# Autodesk Inventor assembly: RA-Manager_Controller
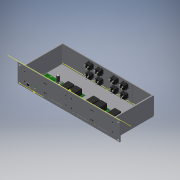
[picture p0: Inventor's stored thumbnail of the model, 180x180]
Saved by Autodesk Inventor 2019.4 (Build 234330000, 330)
## iProperties
Company: Open CASCADE
Created: 2020-03-09
Part Number: RA-Manager_Controller
Material: Genérico
Description: Open CASCADE Model
Document SubType Name: Assembly
Designer: caio.santos
Authority: Unknown
Title: Open CASCADE Shape Model
Author: Author
## Documents named in this file (38)
- C:\Users\caiom\Desktop\Ra-Manager_Mecanica\RA-Manager_Montagem.iam
- C:\Users\caiom\Desktop\Ra-Manager_Mecanica\Ra-Manager_Painel_Frontal.ipt
- C:\Users\caiom\Desktop\Ra-Manager_Mecanica\Ra-Manager_Base.ipt
- C:\Users\caiom\Desktop\Ra-Manager_Mecanica\Ra-Manager_Painel_Traseiro.ipt
- C:\Users\caiom\Desktop\Ra-Manager_Mecanica\Ra-Manager_Painel_Superior.ipt
- C:\Users\caiom\Desktop\Ra-Manager_Mecanica\Ra-Manager_Montagem_Controller.iam
- C:\Users\caiom\Desktop\Ra-Manager_Mecanica\Ra-Manager_Montagem_Relays.iam
- C:\Users\caiom\Desktop\Ra-Manager_Mecanica\Ra-Manager_Painel-Placas_Tras_Cego.ipt
- C:\Users\caiom\Desktop\Ra-Manager_Mecanica\Ra-Manager_Montagem_Plugs.iam
- C:\Users\caiom\Desktop\Ra-Manager_Mecanica\Espacador_Placas.ipt
- C:\Users\caiom\Desktop\Ra-Manager_Mecanica\RA-Manager_Montagem\Design Accelerator\Conexão aparafusada9.iam
- C:\Users\caiom\Desktop\Ra-Manager_Mecanica\RA-Manager_Montagem\Design Accelerator\Conexão aparafusada10.iam
- C:\Users\caiom\Desktop\Ra-Manager_Mecanica\RA-Manager_Montagem\Design Accelerator\Conexão aparafusada11.iam
- C:\Users\caiom\Desktop\Ra-Manager_Mecanica\RA-Manager_Montagem\Design Accelerator\Conexão aparafusada12.iam
- C:\Users\caiom\Desktop\Ra-Manager_Mecanica\RA-Manager_Montagem\Design Accelerator\Conexão aparafusada13.iam
- C:\Users\caiom\Desktop\Ra-Manager_Mecanica\RA-Manager_Montagem\Design Accelerator\Conexão aparafusada14.iam
- C:\Users\caiom\Desktop\Ra-Manager_Mecanica\RA-Manager_Montagem\Design Accelerator\Conexão aparafusada15.iam
- C:\Users\caiom\Desktop\Ra-Manager_Mecanica\RA-Manager_Montagem\Design Accelerator\Conexão aparafusada16.iam
- C:\Users\caiom\Desktop\Ra-Manager_Mecanica\RA-Manager_Montagem\Design Accelerator\Conexão aparafusada17.iam
- C:\Users\caiom\Desktop\Ra-Manager_Mecanica\RA-Manager_Montagem\Design Accelerator\Conexão aparafusada18.iam
- C:\Users\caiom\Desktop\Ra-Manager_Mecanica\RA-Manager_Montagem\Design Accelerator\Conexão aparafusada19.iam
- C:\Users\caiom\Desktop\Ra-Manager_Mecanica\RA-Manager_Montagem\Design Accelerator\Conexão aparafusada20.iam
- C:\Users\caiom\Desktop\Ra-Manager_Mecanica\RA-Manager_Montagem\Design Accelerator\Conexão aparafusada21.iam
- C:\Users\caiom\Desktop\Ra-Manager_Mecanica\RA-Manager_Montagem\Design Accelerator\Conexão aparafusada22.iam
- C:\Users\caiom\Desktop\Ra-Manager_Mecanica\RA-Manager_Montagem\Design Accelerator\Conexão aparafusada23.iam
- C:\Users\caiom\Desktop\Ra-Manager_Mecanica\RA-Manager_Montagem\Design Accelerator\Conexão aparafusada24.iam
- C:\Users\caiom\Desktop\Ra-Manager_Mecanica\RA-Manager_Montagem\Design Accelerator\Conexão aparafusada25.iam
- C:\Users\caiom\Desktop\Ra-Manager_Mecanica\RA-Manager_Montagem\Design Accelerator\Conexão aparafusada26.iam
- C:\Users\caiom\Desktop\Ra-Manager_Mecanica\RA-Manager_Montagem\Design Accelerator\Conexão aparafusada27.iam
- C:\Users\caiom\Desktop\Ra-Manager_Mecanica\RA-Manager_Montagem\Design Accelerator\Conexão aparafusada28.iam
- C:\Users\caiom\Desktop\Ra-Manager_Mecanica\RA-Manager_Montagem\Design Accelerator\Conexão aparafusada29.iam
- C:\Users\caiom\Desktop\Ra-Manager_Mecanica\RA-Manager_Montagem\Design Accelerator\Conexão aparafusada30.iam
- C:\Users\caiom\Desktop\Ra-Manager_Mecanica\RA-Manager_Montagem\Design Accelerator\Conexão aparafusada31.iam
- C:\Users\caiom\Desktop\Ra-Manager_Mecanica\RA-Manager_Montagem\Design Accelerator\Conexão aparafusada32.iam
- C:\Users\caiom\Desktop\Ra-Manager_Mecanica\RA-Manager_Montagem\Design Accelerator\Conexão aparafusada33.iam
- C:\Users\caiom\Desktop\Ra-Manager_Mecanica\RA-Manager_Montagem\Design Accelerator\Conexão aparafusada34.iam
- C:\Users\caiom\Desktop\Ra-Manager_Mecanica\RA-Manager_Montagem\Design Accelerator\Conexão aparafusada35.iam
- C:\Users\caiom\Desktop\Ra-Manager_Mecanica\RA-Manager_Montagem\Design Accelerator\Conexão aparafusada36.iam
## Components (56 placed, 10 different names)
1. Ra-Manager_Painel_Frontal:1 — Coincidência:3, Alinhamento:2, Coincidência:4, Alinhamento:7, Coincidência:12, Coincidência:16, Alinhamento:9, Coincidência:23, Coincidência:24, Coincidência:25, Coincidência:42, Coincidência:44, Coincidência:61, Coincidência:62, Coincidência:100, Coincidência:102, Coincidência:104, Coincidência:106, Coincidência:108, Coincidência:110, Coincidência:112, Coincidência:114, Coincidência:116, Coincidência:118, Coincidência:120, Coincidência:122
2. Ra-Manager_Base:1 — Alinhamento:2, Coincidência:4, Coincidência:7, Coincidência:10, Alinhamento:7, Alinhamento:8, Coincidência:13, Alinhamento:10, Alinhamento:11, Coincidência:29, Coincidência:49, Coincidência:50, Coincidência:51, Coincidência:52, Coincidência:53, Coincidência:54, Coincidência:55, Coincidência:56, Coincidência:57, Coincidência:58, Coincidência:59, Coincidência:60, Coincidência:63, Coincidência:64, Coincidência:65, Coincidência:66, Coincidência:67, Coincidência:68, Coincidência:69, Coincidência:70, Coincidência:71, Coincidência:72, Coincidência:73, Coincidência:74, Coincidência:75, Coincidência:76, Coincidência:77, Coincidência:78, Coincidência:79, Coincidência:80, Coincidência:81, Coincidência:82, Coincidência:83, Coincidência:84, Coincidência:85, Coincidência:86, Coincidência:87, Coincidência:88, Coincidência:89, Coincidência:90, Coincidência:91, Coincidência:92, Coincidência:93, Coincidência:94, Coincidência:95, Coincidência:96, Coincidência:97, Coincidência:98
3. Ra-Manager_Painel_Traseiro:1 — Alinhamento:10, Alinhamento:11, Coincidência:29, Coincidência:30, Coincidência:31, Coincidência:32, Coincidência:33, Coincidência:34, Coincidência:35, Coincidência:36, Coincidência:38, Coincidência:39, Coincidência:40, Coincidência:41
4. Ra-Manager_Painel_Superior:1 — Alinhamento:8, Coincidência:12, Coincidência:13
5. Ra-Manager_Montagem_Controller:1 [sub-assembly] — Alinhamento:9, Coincidência:61, Coincidência:62, Coincidência:99, Coincidência:101, Coincidência:103, Coincidência:105
6. Ra-Manager_Montagem_Relays:1 [sub-assembly] — Coincidência:16, Coincidência:107, Coincidência:109, Coincidência:111, Coincidência:113
7. Ra-Manager_Montagem_Relays:2 [sub-assembly] — Coincidência:23, Coincidência:24, Coincidência:25, Coincidência:43, Coincidência:115, Coincidência:117, Coincidência:119, Coincidência:121
8. Ra-Manager_Montagem_Relays:3 [sub-assembly] — Coincidência:42, Coincidência:43, Coincidência:44
9. Ra-Manager_Painel-Placas_Tras_Cego:1 — Coincidência:30, Coincidência:31, Coincidência:32, Coincidência:37
10. Ra-Manager_Montagem_Plugs:1 [sub-assembly] — Coincidência:33, Coincidência:34, Coincidência:35
11. Ra-Manager_Montagem_Plugs:2 [sub-assembly] — Coincidência:36, Coincidência:37, Coincidência:38
12. Ra-Manager_Painel-Placas_Tras_Cego:2 — Coincidência:39, Coincidência:40, Coincidência:41
13. Espacador_Placas:1 — Coincidência:64
14. Espacador_Placas:2 — Coincidência:65
15. Espacador_Placas:3 — Coincidência:66
16. Espacador_Placas:4 — Coincidência:63
17. Espacador_Placas:5 — Coincidência:52
18. Espacador_Placas:6 — Coincidência:49
19. Espacador_Placas:7 — Coincidência:51
20. Espacador_Placas:8 — Coincidência:50
21. Espacador_Placas:9 — Coincidência:56
22. Espacador_Placas:10 — Coincidência:54
23. Espacador_Placas:11 — Coincidência:55
24. Espacador_Placas:12 — Coincidência:53
25. Espacador_Placas:13 — Coincidência:59
26. Espacador_Placas:14 — Coincidência:57
27. Espacador_Placas:15 — Coincidência:60
28. Espacador_Placas:16 — Coincidência:58
29. Conexão aparafusada:1 [sub-assembly] — Coincidência:67, Coincidência:68
30. Conexão aparafusada:2 [sub-assembly] — Coincidência:69, Coincidência:70
31. Conexão aparafusada:3 [sub-assembly] — Coincidência:71, Coincidência:72
32. Conexão aparafusada:4 [sub-assembly] — Coincidência:73, Coincidência:74
33. Conexão aparafusada:5 [sub-assembly] — Coincidência:75, Coincidência:76
34. Conexão aparafusada:6 [sub-assembly] — Coincidência:77, Coincidência:78
35. Conexão aparafusada:7 [sub-assembly] — Coincidência:79, Coincidência:80
36. Conexão aparafusada:8 [sub-assembly] — Coincidência:81, Coincidência:82
37. Conexão aparafusada:9 [sub-assembly] — Coincidência:83, Coincidência:84
38. Conexão aparafusada:10 [sub-assembly] — Coincidência:85, Coincidência:86
39. Conexão aparafusada:11 [sub-assembly] — Coincidência:87, Coincidência:88
40. Conexão aparafusada:12 [sub-assembly] — Coincidência:89, Coincidência:90
41. Conexão aparafusada:13 [sub-assembly] — Coincidência:91, Coincidência:92
42. Conexão aparafusada:14 [sub-assembly] — Coincidência:93, Coincidência:94
43. Conexão aparafusada:15 [sub-assembly] — Coincidência:95, Coincidência:96
44. Conexão aparafusada:16 [sub-assembly] — Coincidência:97, Coincidência:98
45. Conexão aparafusada:17 [sub-assembly] — Coincidência:99, Coincidência:100
46. Conexão aparafusada:18 [sub-assembly] — Coincidência:101, Coincidência:102
47. Conexão aparafusada:19 [sub-assembly] — Coincidência:103, Coincidência:104
48. Conexão aparafusada:20 [sub-assembly] — Coincidência:105, Coincidência:106
49. Conexão aparafusada:21 [sub-assembly] — Coincidência:107, Coincidência:108
50. Conexão aparafusada:22 [sub-assembly] — Coincidência:109, Coincidência:110
51. Conexão aparafusada:23 [sub-assembly] — Coincidência:111, Coincidência:112
52. Conexão aparafusada:24 [sub-assembly] — Coincidência:113, Coincidência:114
53. Conexão aparafusada:25 [sub-assembly] — Coincidência:115, Coincidência:116
54. Conexão aparafusada:26 [sub-assembly] — Coincidência:117, Coincidência:118
55. Conexão aparafusada:27 [sub-assembly] — Coincidência:119, Coincidência:120
56. Conexão aparafusada:28 [sub-assembly] — Coincidência:121, Coincidência:122
## Relationships (107: Mate 101, Flush 6)
- Coincidência:3 [Mate]: Ra-Manager_Painel_Frontal:1
- Alinhamento:2 [Flush]: Ra-Manager_Painel_Frontal:1 ↔ Ra-Manager_Base:1
- Coincidência:4 [Mate]: Ra-Manager_Painel_Frontal:1 ↔ Ra-Manager_Base:1
- Coincidência:7 [Mate]: Ra-Manager_Base:1
- Coincidência:10 [Mate]: Ra-Manager_Base:1
- Coincidência:11 [Mate] (180 mm)
- Alinhamento:7 [Flush]: Ra-Manager_Painel_Frontal:1 ↔ Ra-Manager_Base:1
- Alinhamento:8 [Flush]: Ra-Manager_Base:1 ↔ Ra-Manager_Painel_Superior:1
- Coincidência:12 [Mate]: Ra-Manager_Painel_Frontal:1 ↔ Ra-Manager_Painel_Superior:1
- Coincidência:13 [Mate]: Ra-Manager_Base:1 ↔ Ra-Manager_Painel_Superior:1
- Coincidência:16 [Mate]: Ra-Manager_Painel_Frontal:1 ↔ Ra-Manager_Montagem_Relays:1
- Alinhamento:9 [Flush]: Ra-Manager_Painel_Frontal:1 ↔ Ra-Manager_Montagem_Controller:1
- Coincidência:23 [Mate]: Ra-Manager_Painel_Frontal:1 ↔ Ra-Manager_Montagem_Relays:2
- Coincidência:24 [Mate]: Ra-Manager_Painel_Frontal:1 ↔ Ra-Manager_Montagem_Relays:2
- Coincidência:25 [Mate]: Ra-Manager_Painel_Frontal:1 ↔ Ra-Manager_Montagem_Relays:2
- Alinhamento:10 [Flush]: Ra-Manager_Base:1 ↔ Ra-Manager_Painel_Traseiro:1
- Alinhamento:11 [Flush]: Ra-Manager_Base:1 ↔ Ra-Manager_Painel_Traseiro:1
- Coincidência:29 [Mate]: Ra-Manager_Base:1 ↔ Ra-Manager_Painel_Traseiro:1
- Coincidência:30 [Mate]: Ra-Manager_Painel_Traseiro:1 ↔ Ra-Manager_Painel-Placas_Tras_Cego:1
- Coincidência:31 [Mate]: Ra-Manager_Painel_Traseiro:1 ↔ Ra-Manager_Painel-Placas_Tras_Cego:1
- Coincidência:32 [Mate]: Ra-Manager_Painel_Traseiro:1 ↔ Ra-Manager_Painel-Placas_Tras_Cego:1
- Coincidência:33 [Mate]: Ra-Manager_Painel_Traseiro:1 ↔ Ra-Manager_Montagem_Plugs:1
- Coincidência:34 [Mate]: Ra-Manager_Painel_Traseiro:1 ↔ Ra-Manager_Montagem_Plugs:1
- Coincidência:35 [Mate]: Ra-Manager_Painel_Traseiro:1 ↔ Ra-Manager_Montagem_Plugs:1
- Coincidência:36 [Mate]: Ra-Manager_Painel_Traseiro:1 ↔ Ra-Manager_Montagem_Plugs:2
- Coincidência:37 [Mate]: Ra-Manager_Painel-Placas_Tras_Cego:1 ↔ Ra-Manager_Montagem_Plugs:2
- Coincidência:38 [Mate]: Ra-Manager_Painel_Traseiro:1 ↔ Ra-Manager_Montagem_Plugs:2
- Coincidência:39 [Mate]: Ra-Manager_Painel_Traseiro:1 ↔ Ra-Manager_Painel-Placas_Tras_Cego:2
- Coincidência:40 [Mate]: Ra-Manager_Painel_Traseiro:1 ↔ Ra-Manager_Painel-Placas_Tras_Cego:2
- Coincidência:41 [Mate]: Ra-Manager_Painel_Traseiro:1 ↔ Ra-Manager_Painel-Placas_Tras_Cego:2
- Coincidência:42 [Mate]: Ra-Manager_Painel_Frontal:1 ↔ Ra-Manager_Montagem_Relays:3
- Coincidência:43 [Mate]: Ra-Manager_Montagem_Relays:2 ↔ Ra-Manager_Montagem_Relays:3
- Coincidência:44 [Mate]: Ra-Manager_Painel_Frontal:1 ↔ Ra-Manager_Montagem_Relays:3
- Coincidência:49 [Mate]: Ra-Manager_Base:1 ↔ Espacador_Placas:6
- Coincidência:50 [Mate]: Ra-Manager_Base:1 ↔ Espacador_Placas:8
- Coincidência:51 [Mate]: Ra-Manager_Base:1 ↔ Espacador_Placas:7
- Coincidência:52 [Mate]: Ra-Manager_Base:1 ↔ Espacador_Placas:5
- Coincidência:53 [Mate]: Ra-Manager_Base:1 ↔ Espacador_Placas:12
- Coincidência:54 [Mate]: Ra-Manager_Base:1 ↔ Espacador_Placas:10
- Coincidência:55 [Mate]: Ra-Manager_Base:1 ↔ Espacador_Placas:11
- Coincidência:56 [Mate]: Ra-Manager_Base:1 ↔ Espacador_Placas:9
- Coincidência:57 [Mate]: Ra-Manager_Base:1 ↔ Espacador_Placas:14
- Coincidência:58 [Mate]: Ra-Manager_Base:1 ↔ Espacador_Placas:16
- Coincidência:59 [Mate]: Ra-Manager_Base:1 ↔ Espacador_Placas:13
- Coincidência:60 [Mate]: Ra-Manager_Base:1 ↔ Espacador_Placas:15
- Coincidência:61 [Mate]: Ra-Manager_Painel_Frontal:1 ↔ Ra-Manager_Montagem_Controller:1
- Coincidência:62 [Mate]: Ra-Manager_Painel_Frontal:1 ↔ Ra-Manager_Montagem_Controller:1
- Coincidência:63 [Mate]: Ra-Manager_Base:1 ↔ Espacador_Placas:4
- Coincidência:64 [Mate]: Ra-Manager_Base:1 ↔ Espacador_Placas:1
- Coincidência:65 [Mate]: Ra-Manager_Base:1 ↔ Espacador_Placas:2
- Coincidência:66 [Mate]: Ra-Manager_Base:1 ↔ Espacador_Placas:3
- Coincidência:67 [Mate]: Ra-Manager_Base:1 ↔ Conexão aparafusada:1
- Coincidência:68 [Mate]: Ra-Manager_Base:1 ↔ Conexão aparafusada:1
- Coincidência:69 [Mate]: Ra-Manager_Base:1 ↔ Conexão aparafusada:2
- Coincidência:70 [Mate]: Ra-Manager_Base:1 ↔ Conexão aparafusada:2
- Coincidência:71 [Mate]: Ra-Manager_Base:1 ↔ Conexão aparafusada:3
- Coincidência:72 [Mate]: Ra-Manager_Base:1 ↔ Conexão aparafusada:3
- Coincidência:73 [Mate]: Ra-Manager_Base:1 ↔ Conexão aparafusada:4
- Coincidência:74 [Mate]: Ra-Manager_Base:1 ↔ Conexão aparafusada:4
- Coincidência:75 [Mate]: Ra-Manager_Base:1 ↔ Conexão aparafusada:5
- Coincidência:76 [Mate]: Ra-Manager_Base:1 ↔ Conexão aparafusada:5
- Coincidência:77 [Mate]: Ra-Manager_Base:1 ↔ Conexão aparafusada:6
- Coincidência:78 [Mate]: Ra-Manager_Base:1 ↔ Conexão aparafusada:6
- Coincidência:79 [Mate]: Ra-Manager_Base:1 ↔ Conexão aparafusada:7
- Coincidência:80 [Mate]: Ra-Manager_Base:1 ↔ Conexão aparafusada:7
- Coincidência:81 [Mate]: Ra-Manager_Base:1 ↔ Conexão aparafusada:8
- Coincidência:82 [Mate]: Ra-Manager_Base:1 ↔ Conexão aparafusada:8
- Coincidência:83 [Mate]: Ra-Manager_Base:1 ↔ Conexão aparafusada:9
- Coincidência:84 [Mate]: Ra-Manager_Base:1 ↔ Conexão aparafusada:9
- Coincidência:85 [Mate]: Ra-Manager_Base:1 ↔ Conexão aparafusada:10
- Coincidência:86 [Mate]: Ra-Manager_Base:1 ↔ Conexão aparafusada:10
- Coincidência:87 [Mate]: Ra-Manager_Base:1 ↔ Conexão aparafusada:11
- Coincidência:88 [Mate]: Ra-Manager_Base:1 ↔ Conexão aparafusada:11
- Coincidência:89 [Mate]: Ra-Manager_Base:1 ↔ Conexão aparafusada:12
- Coincidência:90 [Mate]: Ra-Manager_Base:1 ↔ Conexão aparafusada:12
- Coincidência:91 [Mate]: Ra-Manager_Base:1 ↔ Conexão aparafusada:13
- Coincidência:92 [Mate]: Ra-Manager_Base:1 ↔ Conexão aparafusada:13
- Coincidência:93 [Mate]: Ra-Manager_Base:1 ↔ Conexão aparafusada:14
- Coincidência:94 [Mate]: Ra-Manager_Base:1 ↔ Conexão aparafusada:14
- Coincidência:95 [Mate]: Ra-Manager_Base:1 ↔ Conexão aparafusada:15
- Coincidência:96 [Mate]: Ra-Manager_Base:1 ↔ Conexão aparafusada:15
- Coincidência:97 [Mate]: Ra-Manager_Base:1 ↔ Conexão aparafusada:16
- Coincidência:98 [Mate]: Ra-Manager_Base:1 ↔ Conexão aparafusada:16
- Coincidência:99 [Mate]: Ra-Manager_Montagem_Controller:1 ↔ Conexão aparafusada:17
- Coincidência:100 [Mate]: Ra-Manager_Painel_Frontal:1 ↔ Conexão aparafusada:17
- Coincidência:101 [Mate]: Ra-Manager_Montagem_Controller:1 ↔ Conexão aparafusada:18
- Coincidência:102 [Mate]: Ra-Manager_Painel_Frontal:1 ↔ Conexão aparafusada:18
- Coincidência:103 [Mate]: Ra-Manager_Montagem_Controller:1 ↔ Conexão aparafusada:19
- Coincidência:104 [Mate]: Ra-Manager_Painel_Frontal:1 ↔ Conexão aparafusada:19
- Coincidência:105 [Mate]: Ra-Manager_Montagem_Controller:1 ↔ Conexão aparafusada:20
- Coincidência:106 [Mate]: Ra-Manager_Painel_Frontal:1 ↔ Conexão aparafusada:20
- Coincidência:107 [Mate]: Ra-Manager_Montagem_Relays:1 ↔ Conexão aparafusada:21
- Coincidência:108 [Mate]: Ra-Manager_Painel_Frontal:1 ↔ Conexão aparafusada:21
- Coincidência:109 [Mate]: Ra-Manager_Montagem_Relays:1 ↔ Conexão aparafusada:22
- Coincidência:110 [Mate]: Ra-Manager_Painel_Frontal:1 ↔ Conexão aparafusada:22
- Coincidência:111 [Mate]: Ra-Manager_Montagem_Relays:1 ↔ Conexão aparafusada:23
- Coincidência:112 [Mate]: Ra-Manager_Painel_Frontal:1 ↔ Conexão aparafusada:23
- Coincidência:113 [Mate]: Ra-Manager_Montagem_Relays:1 ↔ Conexão aparafusada:24
- Coincidência:114 [Mate]: Ra-Manager_Painel_Frontal:1 ↔ Conexão aparafusada:24
- Coincidência:115 [Mate]: Ra-Manager_Montagem_Relays:2 ↔ Conexão aparafusada:25
- Coincidência:116 [Mate]: Ra-Manager_Painel_Frontal:1 ↔ Conexão aparafusada:25
- Coincidência:117 [Mate]: Ra-Manager_Montagem_Relays:2 ↔ Conexão aparafusada:26
- Coincidência:118 [Mate]: Ra-Manager_Painel_Frontal:1 ↔ Conexão aparafusada:26
- Coincidência:119 [Mate]: Ra-Manager_Montagem_Relays:2 ↔ Conexão aparafusada:27
- Coincidência:120 [Mate]: Ra-Manager_Painel_Frontal:1 ↔ Conexão aparafusada:27
- Coincidência:121 [Mate]: Ra-Manager_Montagem_Relays:2 ↔ Conexão aparafusada:28
- Coincidência:122 [Mate]: Ra-Manager_Painel_Frontal:1 ↔ Conexão aparafusada:28
